# Autodesk Inventor assembly: ring+GEARASS
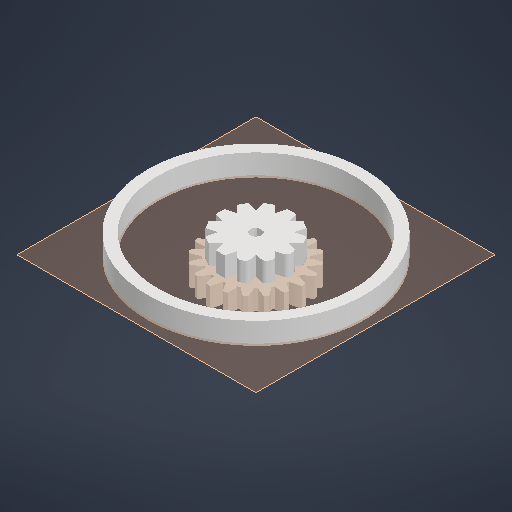
[picture p0: Inventor's stored thumbnail of the model, 512x512]
Saved by Autodesk Inventor 2027.1 (Build 311267000, 267)
## iProperties
Created: 2026-10-02
Part Number: ring+GEARASS
Document SubType Name: Assembly
Designer: HP
Author: HP
## Documents named in this file (3)
- C:\Users\HP\Documents\GitHub\Robotic-arm\3dfiles\ring+GEARASS.iam
- C:\Users\HP\Documents\GitHub\Robotic-arm\3dfiles\ringGEAR.ipt
- C:\Users\HP\Documents\GitHub\Robotic-arm\3dfiles\ring+GEARASS\Design Accelerator\Spur Gears1.iam
## Components (2 placed, 2 different names)
1. ringGEAR:1 — Mate:1, Mate:2
2. Spur Gears:1 [sub-assembly] — Mate:1, Mate:2
## Relationships (2: Mate 2)
- Mate:1: ringGEAR:1 ↔ Spur Gears:1
- Mate:2: ringGEAR:1 ↔ Spur Gears:1
